# Autodesk Inventor assembly: Full mount
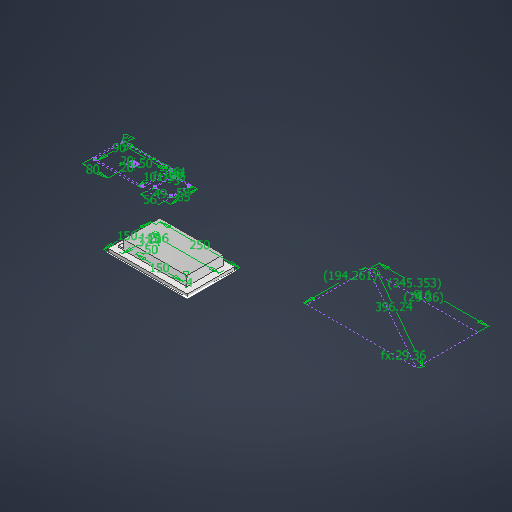
[picture p0: Inventor's stored thumbnail of the model, 512x512]
Saved by Autodesk Inventor 2025.1 (Build 291241000, 241)
## iProperties
Created: 2025-02-09
Part Number: Full mount
Document SubType Name: Assembly
Designer: jerem
Author: jerem
## Documents named in this file (3)
- C:\Users\jerem\Documents\GitHub\Perovskite-Automated-Synthesis-System\CAD\Object Mounts\Full mount.iam
- C:\Users\jerem\Documents\GitHub\Perovskite-Automated-Synthesis-System\CAD\Object Mounts\Main Mount.ipt
- C:\Users\jerem\Documents\GitHub\Perovskite-Automated-Synthesis-System\CAD\Non 3D Printed Parts\Stepper Power Supply.ipt
## Components (2 placed, 2 different names)
1. Main Mount:1 — Mate:1, Mate:2, Mate:3
2. Stepper Power Supply:1 — Mate:1, Mate:2, Mate:3
## Relationships (3: Mate 3)
- Mate:1: Main Mount:1 ↔ Stepper Power Supply:1
- Mate:2: Main Mount:1 ↔ Stepper Power Supply:1
- Mate:3: Main Mount:1 ↔ Stepper Power Supply:1
